# Autodesk Inventor assembly: HS-311 Hitec Standard Servo and Horn
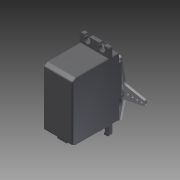
[picture p0: Inventor's stored thumbnail of the model, 180x180]
Saved by Autodesk Inventor 2012 (Build 160160000, 160)
## iProperties
Created: 2011-06-28
Part Number: HS-311 Hitec Standard Servo and Horn
Document SubType Name: Assembly
Designer: Byron
## Documents named in this file (4)
- C:\Users\Nano\Documents\InventorByron\InventorMasterProject\Imported Components\HS-311 Hitec Standard Servo and Horn\HS-311 Hitec Standard Servo and Horn.iam
- C:\Users\Nano\Documents\InventorByron\InventorMasterProject\Imported Components\HS-311 Hitec Standard Servo and Horn\HS-311 Hitec Standard Servo.ipt
- C:\Users\Nano\Documents\InventorByron\InventorMasterProject\Imported Components\HS-311 Hitec Standard Servo and Horn\#4 Screw.ipt
- C:\Users\Nano\Documents\InventorByron\InventorMasterProject\standardServo\servoHornX.ipt
## Components (3 placed, 3 different names)
1. HS-311 Hitec Standard Servo:1 — Mate:5, Mate:6
2. Servo Horn:1 — Mate:5, Mate:6, Mate:7, Mate:8
3. #4 Screw:1 — Mate:7, Mate:8
## Relationships (4: Mate 4)
- Mate:5: HS-311 Hitec Standard Servo:1 ↔ Servo Horn:1
- Mate:6: HS-311 Hitec Standard Servo:1 ↔ Servo Horn:1
- Mate:7: Servo Horn:1 ↔ #4 Screw:1
- Mate:8: Servo Horn:1 ↔ #4 Screw:1
